# Autodesk Inventor assembly: Bearing Cart
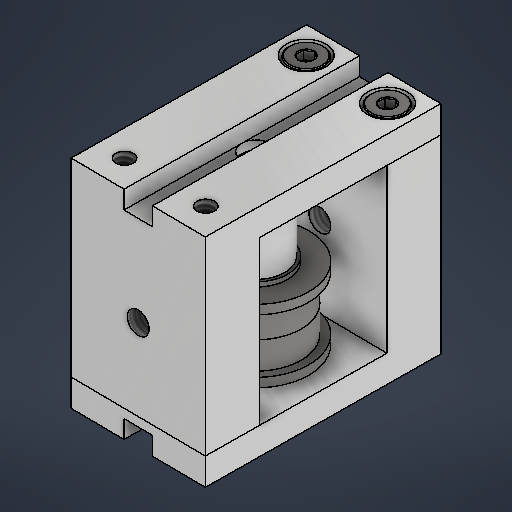
[picture p0: Inventor's stored thumbnail of the model, 512x512]
Saved by Autodesk Inventor 2026 (Build 300175050, 175E)
## iProperties
Created: 2025-05-26
Part Number: Bearing Cart
Document SubType Name: Assembly
Designer: Joshua Eah
Author: Joshua Eah
## Documents named in this file (5)
- C:\Users\Joshua Eah\Documents\GitHub\Voron-0\CAD\Tulip - Machined Parts\Idlers\Bearing Cart.iam
- C:\Users\Joshua Eah\Documents\GitHub\Voron-0\CAD\Tulip - Machined Parts\Idlers\Bearing Sled.ipt
- C:\Users\Joshua Eah\Documents\GitHub\Voron-0\CAD\Master Assembly\Hardware\F623 Stack.iam
- C:\Users\Joshua Eah\Documents\GitHub\Voron-0\CAD\Master Assembly\Hardware\M2x6 SHCS.ipt
- C:\Users\Joshua Eah\Documents\GitHub\Voron-0\CAD\Machined Parts\Spacers\Spacer.ipt
## Components (8 placed, 4 different names)
1. Bearing Sled:1 — Insert:1, Insert:3, Insert:4, Insert:8, Insert:9
2. Bearing Sled:2 — Insert:1, Insert:5, Insert:6, Insert:7, Insert:9
3. F623 Stack:1 [sub-assembly] — Insert:7
4. M2x6 SHCS:1 — Insert:3
5. M2x6 SHCS:2 — Insert:4
6. M2x6 SHCS:3 — Insert:5
7. M2x6 SHCS:4 — Insert:6
8. Spacer:1 — Insert:8
## Relationships (8: Insert 8)
- Insert:1: Bearing Sled:1 ↔ Bearing Sled:2
- Insert:3: Bearing Sled:1 ↔ M2x6 SHCS:1
- Insert:4: Bearing Sled:1 ↔ M2x6 SHCS:2
- Insert:5: Bearing Sled:2 ↔ M2x6 SHCS:3
- Insert:6: Bearing Sled:2 ↔ M2x6 SHCS:4
- Insert:7: Bearing Sled:2 ↔ F623 Stack:1
- Insert:8: Bearing Sled:1 ↔ Spacer:1
- Insert:9: Bearing Sled:1 ↔ Bearing Sled:2
